# Autodesk Inventor assembly: motor_w_gear
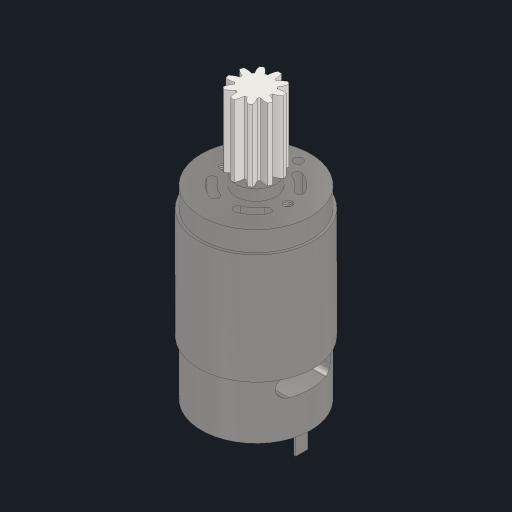
[picture p0: Inventor's stored thumbnail of the model, 512x512]
Saved by Autodesk Inventor 2023 (Build 270158000, 158)
## iProperties
Created: 2024-04-29
Part Number: motor_w_gear
Document SubType Name: Assembly
Designer: szymo
Mass: 120 g
Surface Area: 100.129 cm^2
Volume: 27.5535 cm^3
Density: 4.35516 g/cm^3
Author: szymo
## Documents named in this file (3)
- C:\zRozne\roboilo\robots\codename wafel - australia\3d_parts\rev2\motor_w_gear.iam
- C:\zRozne\roboilo\robots\codename wafel - australia\3d_parts\rev2\rs390.ipt
- C:\zRozne\roboilo\robots\codename wafel - australia\3d_parts\rev2\Design Accelerator\rs390_gear.iam
## Components (2 placed, 2 different names)
1. rs390_gear:1 [sub-assembly] — Mate:1, Mate:2
2. rs390:1 — Mate:1, Mate:2
## Relationships (2: Mate 2)
- Mate:1: rs390_gear:1 ↔ rs390:1
- Mate:2 (1 mm): rs390_gear:1 ↔ rs390:1
